# Autodesk Inventor assembly: input_assembly
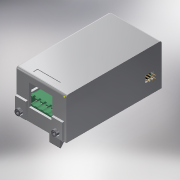
[picture p0: Inventor's stored thumbnail of the model, 180x180]
Saved by Autodesk Inventor 2019 (Build 230136000, 136)
## iProperties
Created: 2020-05-12
Part Number: input_assembly
Document SubType Name: Assembly
Designer: Mateusz
Author: Mateusz
## Documents named in this file (6)
- D:\Projekty\Azure Sphere IoT Controller\Addons\Input\case\input_assembly.iam
- D:\Projekty\Azure Sphere IoT Controller\Addons\Input\case\input.ipt
- D:\Projekty\Azure Sphere IoT Controller\Addons\Input\case\bottom.ipt
- D:\Projekty\Azure Sphere IoT Controller\Addons\Input\case\top.ipt
- D:\Projekty\Azure Sphere IoT Controller\Addons\Input\case\SHCS M3-20.ipt
- D:\Projekty\Azure Sphere IoT Controller\Addons\Input\case\DIN_mount.ipt
## Components (7 placed, 5 different names)
1. input:1 — Mate:1, Mate:2, Mate:3
2. bottom:1 — Mate:1, Mate:2, Mate:3, Mate:4, Mate:5, Mate:6, Mate:13, Mate:14, Mate:15
3. top:1 — Mate:4, Mate:5, Mate:6, Mate:7, Mate:8, Mate:9, Mate:10, Mate:11, Mate:12
4. SHCS M3-20:1 — Mate:7, Mate:12
5. SHCS M3-20:2 — Mate:8, Mate:11
6. SHCS M3-20:3 — Mate:9, Mate:10
7. DIN_mount:1 — Mate:13, Mate:14, Mate:15
## Relationships (15: Mate 15)
- Mate:1: input:1 ↔ bottom:1
- Mate:2: input:1 ↔ bottom:1
- Mate:3: input:1 ↔ bottom:1
- Mate:4: bottom:1 ↔ top:1
- Mate:5: bottom:1 ↔ top:1
- Mate:6: bottom:1 ↔ top:1
- Mate:7: top:1 ↔ SHCS M3-20:1
- Mate:8: top:1 ↔ SHCS M3-20:2
- Mate:9: top:1 ↔ SHCS M3-20:3
- Mate:10: top:1 ↔ SHCS M3-20:3
- Mate:11: top:1 ↔ SHCS M3-20:2
- Mate:12: top:1 ↔ SHCS M3-20:1
- Mate:13: bottom:1 ↔ DIN_mount:1
- Mate:14: bottom:1 ↔ DIN_mount:1
- Mate:15: bottom:1 ↔ DIN_mount:1
